# Autodesk Inventor assembly: Vertical
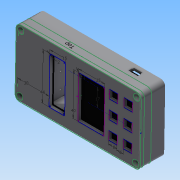
[picture p0: Inventor's stored thumbnail of the model, 180x180]
Saved by Autodesk Inventor 2016 (Build 200138000, 138)
## iProperties
Created: 2016-03-29
Part Number: Vertical
Document SubType Name: Assembly
Designer: admin
Author: admin
## Documents named in this file (9)
- E:\Alex\HS-Spectrophotometer\parts\New vesion\AK-C-C10-Vertical.iam
- E:\Alex\HS-Spectrophotometer\parts\New vesion\AK-C-C10-Left_wall.ipt
- E:\Alex\HS-Spectrophotometer\parts\New vesion\AK-C-C10-Right_wall.ipt
- E:\Alex\HS-Spectrophotometer\parts\New vesion\AK-C-C10-Separator.ipt
- E:\Alex\HS-Spectrophotometer\parts\New vesion\AK-C-C10-Top.ipt
- E:\Alex\HS-Spectrophotometer\parts\New vesion\AK-C-C10-Main-Board.ipt
- E:\Alex\HS-Spectrophotometer\parts\New vesion\AK-C-C10-LED-Board-Assembly.iam
- E:\Alex\HS-Spectrophotometer\parts\New vesion\AK-C-C10-Pinhole-Board.ipt
- E:\Alex\HS-Spectrophotometer\parts\New vesion\AK-C-C10-Sensor-Board.ipt
## Components (10 placed, 8 different names)
1. AK-C-C10-Left_wall:1 — Mate:1, Flush:1, Flush:2, Mate:12, Flush:3, Flush:4, Mate:21, Mate:23, Mate:24
2. AK-C-C10-Right_wall:1 — Mate:1, Flush:1, Flush:2, Mate:12, Flush:3, Flush:4, Mate:13, Mate:22, Mate:29, Mate:30
3. AK-C-C10-Separator:1 — Mate:28, Mate:29, Mate:30, Mate:31, Mate:34, Mate:37, Mate:40
4. AK-C-C10-Separator:2 — Mate:23, Mate:24, Mate:25
5. AK-C-C10-Top:1 — Mate:13, Mate:18, Mate:19, Mate:20, Mate:21, Mate:22, Mate:42, Mate:44, Mate:47, Mate:49
6. AK-C-C10-Main-Board:1 — Mate:18, Mate:19, Mate:20, Mate:25, Mate:28, Mate:43, Mate:45, Mate:46, Mate:48
7. AK-C-C10-LED-Board-Assembly:1 [sub-assembly] — Mate:31, Mate:44, Mate:45
8. AK-C-C10-Pinhole-Board:1 — Mate:34, Mate:46, Mate:47
9. AK-C-C10-Pinhole-Board:2 — Mate:37, Mate:48, Mate:49
10. AK-C-C10-Sensor-Board:1 — Mate:40, Mate:42, Mate:43
## Relationships (30: Mate 26, Flush 4)
- Mate:1: AK-C-C10-Left_wall:1 ↔ AK-C-C10-Right_wall:1
- Flush:1: AK-C-C10-Left_wall:1 ↔ AK-C-C10-Right_wall:1
- Flush:2: AK-C-C10-Left_wall:1 ↔ AK-C-C10-Right_wall:1
- Mate:12: AK-C-C10-Left_wall:1 ↔ AK-C-C10-Right_wall:1
- Flush:3: AK-C-C10-Left_wall:1 ↔ AK-C-C10-Right_wall:1
- Flush:4: AK-C-C10-Left_wall:1 ↔ AK-C-C10-Right_wall:1
- Mate:13: AK-C-C10-Right_wall:1 ↔ AK-C-C10-Top:1
- Mate:18: AK-C-C10-Top:1 ↔ AK-C-C10-Main-Board:1
- Mate:19: AK-C-C10-Top:1 ↔ AK-C-C10-Main-Board:1
- Mate:20: AK-C-C10-Top:1 ↔ AK-C-C10-Main-Board:1
- Mate:21: AK-C-C10-Left_wall:1 ↔ AK-C-C10-Top:1
- Mate:22: AK-C-C10-Right_wall:1 ↔ AK-C-C10-Top:1
- Mate:23 (0.2 mm): AK-C-C10-Left_wall:1 ↔ AK-C-C10-Separator:2
- Mate:24 (0.5 mm): AK-C-C10-Left_wall:1 ↔ AK-C-C10-Separator:2
- Mate:25: AK-C-C10-Separator:2 ↔ AK-C-C10-Main-Board:1
- Mate:28: AK-C-C10-Separator:1 ↔ AK-C-C10-Main-Board:1
- Mate:29 (0.2 mm): AK-C-C10-Right_wall:1 ↔ AK-C-C10-Separator:1
- Mate:30 (0.5 mm): AK-C-C10-Right_wall:1 ↔ AK-C-C10-Separator:1
- Mate:31: AK-C-C10-Separator:1 ↔ AK-C-C10-LED-Board-Assembly:1
- Mate:34: AK-C-C10-Separator:1 ↔ AK-C-C10-Pinhole-Board:1
- Mate:37: AK-C-C10-Separator:1 ↔ AK-C-C10-Pinhole-Board:2
- Mate:40: AK-C-C10-Separator:1 ↔ AK-C-C10-Sensor-Board:1
- Mate:42: AK-C-C10-Top:1 ↔ AK-C-C10-Sensor-Board:1
- Mate:43: AK-C-C10-Main-Board:1 ↔ AK-C-C10-Sensor-Board:1
- Mate:44: AK-C-C10-Top:1 ↔ AK-C-C10-LED-Board-Assembly:1
- Mate:45: AK-C-C10-Main-Board:1 ↔ AK-C-C10-LED-Board-Assembly:1
- Mate:46: AK-C-C10-Main-Board:1 ↔ AK-C-C10-Pinhole-Board:1
- Mate:47: AK-C-C10-Top:1 ↔ AK-C-C10-Pinhole-Board:1
- Mate:48: AK-C-C10-Main-Board:1 ↔ AK-C-C10-Pinhole-Board:2
- Mate:49: AK-C-C10-Top:1 ↔ AK-C-C10-Pinhole-Board:2
